# Autodesk Inventor assembly: TV Mount
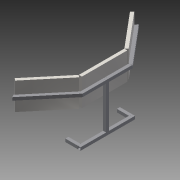
[picture p0: Inventor's stored thumbnail of the model, 180x180]
Saved by Autodesk Inventor 2015 (Build 190159000, 159)
## iProperties
Created: 2016-03-22
Part Number: TV Mount
Document SubType Name: Assembly
Designer: Mac
Author: Mac
## Documents named in this file (6)
- C:\Users\Mac\Desktop\MotionBase\CAD\MotionBaseCAD\TV Mount.iam
- C:\Users\Mac\Desktop\MotionBase\CAD\MotionBaseCAD\tube support base.ipt
- C:\Users\Mac\Desktop\MotionBase\CAD\MotionBaseCAD\Tube support base 2.ipt
- C:\Users\Mac\Desktop\MotionBase\CAD\MotionBaseCAD\sqare vertical.ipt
- C:\Users\Mac\Desktop\MotionBase\CAD\MotionBaseCAD\Television.ipt
- C:\Users\Mac\Desktop\MotionBase\CAD\MotionBaseCAD\TV mount center.ipt
## Components (10 placed, 5 different names)
1. tube support base:1 — Flush:1, Mate:1, Flush:2, Flush:3, Flush:4, Mate:2, Flush:5, Mate:3
2. Tube support base 2:1 — Flush:1, Mate:1, Flush:2, Mate:4
3. Tube support base 2:2 — Flush:3, Flush:4, Mate:2
4. sqare vertical:1 — Flush:5, Mate:3, Mate:4, Mate:13, Flush:10, Flush:11, Flush:12
5. Television:1 — Mate:14, Flush:11, Flush:13, Flush:14, Mate:19
6. Television:2 — Mate:15, Mate:17, Flush:13
7. Television:3 — Mate:16, Mate:18, Flush:14
8. TV mount center:1 — Flush:6, Flush:7, Mate:7, Flush:8, Mate:8, Flush:9, Mate:13, Flush:10, Mate:14, Flush:12, Mate:19, Mate:22, Mate:23
9. TV mount center:2 — Flush:6, Mate:7, Flush:8, Mate:16, Mate:18, Mate:21, Angle:2
10. TV mount center:3 — Flush:7, Mate:8, Flush:9, Mate:15, Mate:17, Mate:20, Angle:1
## Relationships (33: Mate 17, Flush 14, Angle 2)
- Flush:1: tube support base:1 ↔ Tube support base 2:1
- Mate:1: tube support base:1 ↔ Tube support base 2:1
- Flush:2: tube support base:1 ↔ Tube support base 2:1
- Flush:3: tube support base:1 ↔ Tube support base 2:2
- Flush:4: tube support base:1 ↔ Tube support base 2:2
- Mate:2: tube support base:1 ↔ Tube support base 2:2
- Flush:5: tube support base:1 ↔ sqare vertical:1
- Mate:3: tube support base:1 ↔ sqare vertical:1
- Mate:4 (-431.8 mm): Tube support base 2:1 ↔ sqare vertical:1
- Flush:6: TV mount center:1 ↔ TV mount center:2
- Flush:7: TV mount center:1 ↔ TV mount center:3
- Mate:7: TV mount center:1 ↔ TV mount center:2
- Flush:8: TV mount center:1 ↔ TV mount center:2
- Mate:8: TV mount center:1 ↔ TV mount center:3
- Flush:9: TV mount center:1 ↔ TV mount center:3
- Mate:13 (-50.8 mm): sqare vertical:1 ↔ TV mount center:1
- Flush:10: sqare vertical:1 ↔ TV mount center:1
- Mate:14: Television:1 ↔ TV mount center:1
- Mate:15: Television:2 ↔ TV mount center:3
- Mate:16: Television:3 ↔ TV mount center:2
- Flush:11: sqare vertical:1 ↔ Television:1
- Flush:12: sqare vertical:1 ↔ TV mount center:1
- Mate:17: Television:2 ↔ TV mount center:3
- Mate:18: Television:3 ↔ TV mount center:2
- Flush:13: Television:1 ↔ Television:2
- Flush:14: Television:1 ↔ Television:3
- Mate:19: Television:1 ↔ TV mount center:1
- Mate:20: TV mount center:3
- Angle:1 (140 deg): TV mount center:3
- Mate:21: TV mount center:2
- Angle:2 (140 deg): TV mount center:2
- Mate:22: TV mount center:1
- Mate:23: TV mount center:1
